# Autodesk Inventor assembly: ALL
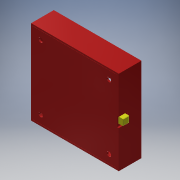
[picture p0: Inventor's stored thumbnail of the model, 180x180]
Saved by Autodesk Inventor 2019 (Build 230136000, 136)
## iProperties
Created: 2018-12-19
Part Number: ALL
Material: Типовые
Document SubType Name: Assembly
Designer: aldanstar
Author: aldanstar
## Documents named in this file (10)
- C:\Users\astarovo\Inventor Projects\ESP8266_DOWNLOADER\ALL.iam
- C:\Users\astarovo\Inventor Projects\ESP8266_DOWNLOADER\BOTTOM.ipt
- C:\Users\astarovo\Inventor Projects\ESP8266_DOWNLOADER\BUTTON_OUTSIDE.ipt
- C:\Users\astarovo\Inventor Projects\ESP8266_DOWNLOADER\BUTTON_INSIDE.ipt
- C:\Users\astarovo\Inventor Projects\ESP8266_DOWNLOADER\BUTTON_TOP.ipt
- C:\Users\astarovo\Inventor Projects\ESP8266_DOWNLOADER\TOP.ipt
- C:\Users\astarovo\Inventor Projects\ESP8266_DOWNLOADER\BUTTON.ipt
- C:\Users\astarovo\Inventor Projects\ESP8266_DOWNLOADER\BUTTON2.ipt
- C:\Users\astarovo\Inventor Projects\ESP8266_DOWNLOADER\LED1.ipt
- C:\Users\astarovo\Inventor Projects\ESP8266_DOWNLOADER\LED2.ipt
## Components (10 placed, 9 different names)
1. BOTTOM:1 — Ползун:1, Цилиндрический:1, Совмещение:2, Жесткий:3, Заподлицо:1, Жесткий:4
2. BUTTON_OUTSIDE:1 — Ползун:1, Обкатка:1
3. BUTTON_INSIDE:1 — Цилиндрический:1, Обкатка:1
4. BUTTON_TOP:1 — Совмещение:2, Жесткий:3
5. TOP:1 — Заподлицо:1, Жесткий:4, Совмещение:3, Совмещение:4, Обкатка:2, Обкатка:3, Ползун:6, Жесткий:5, Жесткий:6
6. BUTTON:1 — Совмещение:3, Обкатка:2
7. BUTTON:2 — Совмещение:4, Обкатка:3
8. BUTTON2:1 — Ползун:6
9. LED1:1 — Жесткий:6
10. LED2:1 — Жесткий:5
## Relationships (14: WeldJoint 4, Transitional 3, Mate 3, TranslationJoint 2, CylindricalJoint 1, Flush 1)
- Ползун:1 [TranslationJoint]: BOTTOM:1 ↔ BUTTON_OUTSIDE:1
- Цилиндрический:1 [CylindricalJoint]: BOTTOM:1 ↔ BUTTON_INSIDE:1
- Обкатка:1 [Transitional]: BUTTON_OUTSIDE:1 ↔ BUTTON_INSIDE:1
- Совмещение:2 [Mate]: BOTTOM:1 ↔ BUTTON_TOP:1
- Жесткий:3 [WeldJoint]: BOTTOM:1 ↔ BUTTON_TOP:1
- Заподлицо:1 [Flush]: BOTTOM:1 ↔ TOP:1
- Жесткий:4 [WeldJoint]: BOTTOM:1 ↔ TOP:1
- Совмещение:3 [Mate]: TOP:1 ↔ BUTTON:1
- Совмещение:4 [Mate]: TOP:1 ↔ BUTTON:2
- Обкатка:2 [Transitional]: TOP:1 ↔ BUTTON:1
- Обкатка:3 [Transitional]: TOP:1 ↔ BUTTON:2
- Ползун:6 [TranslationJoint] (0.1 mm): TOP:1 ↔ BUTTON2:1
- Жесткий:5 [WeldJoint]: TOP:1 ↔ LED2:1
- Жесткий:6 [WeldJoint]: TOP:1 ↔ LED1:1
